# Autodesk Inventor assembly: Drivebox_MIR
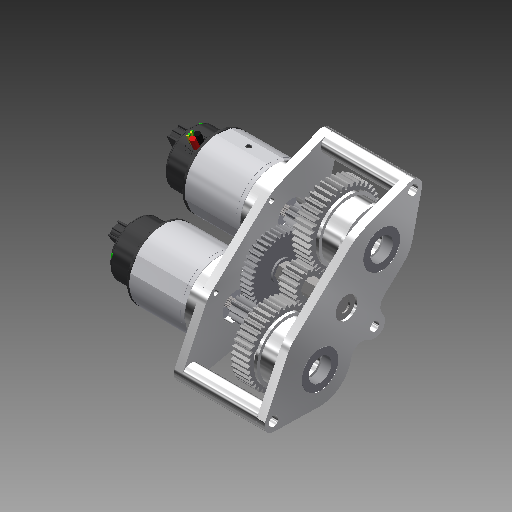
[picture p0: Inventor's stored thumbnail of the model, 512x512]
Saved by Autodesk Inventor 2019.4 (Build 234330000, 330)
## iProperties
Created: 2020-01-05
Part Number: Drivebox_MIR
Document SubType Name: Assembly
Designer: Mark
Mass: 1559.59 g
Surface Area: 2473.44 cm^2
Volume: 631.167 cm^3
Density: 2.47097 g/cm^3
Author: Mark
## Documents named in this file (14)
- C:\Users\admin\Desktop\FRC 2020 Engineering\GitHub\7738-2020\CAD\Gearbox\Drivebox_MIR.iam
- C:\Users\admin\Desktop\FRC 2020 Engineering\GitHub\7738-2020\CAD\Gearbox\Gearbox Plate 1_MIR.ipt
- C:\Users\admin\Desktop\FRC 2020 Engineering\GitHub\7738-2020\CAD\Gearbox\Gearbox Plate 2_MIR.ipt
- C:\Users\admin\Desktop\FRC 2020 Engineering\GitHub\7738-2020\CAD\Gearbox\Shaft Jr_MIR.ipt
- C:\Users\admin\Desktop\FRC 2020 Engineering\GitHub\7738-2020\CAD\Gearbox\F6800_MIR.ipt
- C:\Users\admin\Desktop\FRC 2020 Engineering\GitHub\7738-2020\CAD\Gearbox\Spacer_MIR.ipt
- C:\Users\admin\Desktop\FRC 2020 Engineering\GitHub\7738-2020\CAD\Gearbox\Falcon_500_Powered_by_Talon_FX_217-6515_MIR.ipt
- C:\Users\admin\Desktop\FRC 2020 Engineering\GitHub\7738-2020\CAD\Gearbox\F6804_MIR.ipt
- C:\Users\admin\Desktop\FRC 2020 Engineering\GitHub\7738-2020\CAD\Gearbox\10T_Steel_Spur_Gear_20_DP_12T_Center_Distance_Falcon_Motor_217-6917_MIR.ipt
- C:\Users\admin\Desktop\FRC 2020 Engineering\GitHub\7738-2020\CAD\Gearbox\40t_Aluminum_Spur_Gear_20_DP_1_2_Hex_Bore_217-2708_MIR.ipt
- C:\Users\admin\Desktop\FRC 2020 Engineering\GitHub\7738-2020\CAD\Gearbox\Gearbox\Design Accelerator\Spur Gears1_MIR1.iam
- C:\Users\admin\Desktop\FRC 2020 Engineering\GitHub\7738-2020\CAD\Gearbox\Gearbox\Design Accelerator\Spur Gears2_MIR1.iam
- C:\Users\admin\Desktop\FRC 2020 Engineering\GitHub\7738-2020\CAD\Gearbox\HTD 5M 30 20mm ID Keyed_MIR.ipt
- C:\Users\admin\Desktop\FRC 2020 Engineering\GitHub\7738-2020\CAD\Motor Spacer_MIR.ipt
## Components (21 placed, 13 different names)
1. Gearbox Plate 1_MIR:1 — Flush:3, Mate:4, Mate:3, Mate:45, Mate:47, Mate:46, Mate:14, Mate:13, Mate:18, Mate:17, Mate:16, Mate:15, Mate:25, Mate:26, Mate:43, Mate:54, Mate:56
2. Gearbox Plate 2_MIR:1 — Flush:3, Mate:39, Mate:38, Mate:37, Mate:44, Mate:34, Mate:33, Mate:36, Mate:35, Mate:40, Mate:49, Mate:51
3. Shaft Jr_MIR:1 — Mate:8, Mate:7, Mate:41
4. F6800_MIR:1 — Mate:39, Mate:8, Mate:7, Mate:4, Mate:3, Mate:42
5. F6800_MIR:2 — Mate:41, Mate:38, Mate:37
6. Spacer_MIR:1 — Mate:44, Mate:45
7. Spacer_MIR:2 — Mate:47, Mate:46
8. Spacer_MIR:3 — Mate:14, Mate:13
9. Falcon_500_Powered_by_Talon_FX_217-6515_MIR:1 — Mate:18, Mate:17, Mate:23, Mate:53
10. Falcon_500_Powered_by_Talon_FX_217-6515_MIR:2 — Mate:16, Mate:15, Mate:52, Mate:55
11. F6804_MIR:1 — Mate:34, Mate:33, Mate:31, Mate:50
12. F6804_MIR:2 — Mate:36, Mate:35, Mate:32, Mate:48
13. 10T_Steel_Spur_Gear_20_DP_12T_Center_Distance_Falcon_Motor_217-6917_MIR:1 — Mate:52, Mate:25
14. 10T_Steel_Spur_Gear_20_DP_12T_Center_Distance_Falcon_Motor_217-6917_MIR:2 — Mate:26, Mate:23
15. 40t_Aluminum_Spur_Gear_20_DP_1_2_Hex_Bore_217-2708_MIR:1 — Mate:43, Mate:42, Mate:30
16. Spur Gears1_MIR1:1 [sub-assembly] — Mate:40, Mate:31, Mate:30, Flush:2
17. Spur Gears2_MIR1:1 [sub-assembly] — Flush:2, Mate:32
18. HTD 5M 30 20mm ID Keyed_MIR:1 — Mate:49, Mate:48
19. HTD 5M 30 20mm ID Keyed_MIR:2 — Mate:51, Mate:50
20. Motor Spacer_MIR:1 — Mate:54, Mate:53
21. Motor Spacer_MIR:2 — Mate:56, Mate:55
## Relationships (42: Mate 40, Flush 2)
- Flush:3: Gearbox Plate 1_MIR:1 ↔ Gearbox Plate 2_MIR:1
- Mate:39: Gearbox Plate 2_MIR:1 ↔ F6800_MIR:1
- Mate:8 (0.2 mm): Shaft Jr_MIR:1 ↔ F6800_MIR:1
- Mate:7: Shaft Jr_MIR:1 ↔ F6800_MIR:1
- Mate:4: Gearbox Plate 1_MIR:1 ↔ F6800_MIR:1
- Mate:3: Gearbox Plate 1_MIR:1 ↔ F6800_MIR:1
- Mate:41 (0.2 mm): Shaft Jr_MIR:1 ↔ F6800_MIR:2
- Mate:38: Gearbox Plate 2_MIR:1 ↔ F6800_MIR:2
- Mate:37: Gearbox Plate 2_MIR:1 ↔ F6800_MIR:2
- Mate:44: Gearbox Plate 2_MIR:1 ↔ Spacer_MIR:1
- Mate:45: Gearbox Plate 1_MIR:1 ↔ Spacer_MIR:1
- Mate:47: Gearbox Plate 1_MIR:1 ↔ Spacer_MIR:2
- Mate:46: Gearbox Plate 1_MIR:1 ↔ Spacer_MIR:2
- Mate:14: Gearbox Plate 1_MIR:1 ↔ Spacer_MIR:3
- Mate:13: Gearbox Plate 1_MIR:1 ↔ Spacer_MIR:3
- Mate:18 (7.5 mm): Gearbox Plate 1_MIR:1 ↔ Falcon_500_Powered_by_Talon_FX_217-6515_MIR:1
- Mate:17: Gearbox Plate 1_MIR:1 ↔ Falcon_500_Powered_by_Talon_FX_217-6515_MIR:1
- Mate:16 (7.5 mm): Gearbox Plate 1_MIR:1 ↔ Falcon_500_Powered_by_Talon_FX_217-6515_MIR:2
- Mate:15: Gearbox Plate 1_MIR:1 ↔ Falcon_500_Powered_by_Talon_FX_217-6515_MIR:2
- Mate:34: Gearbox Plate 2_MIR:1 ↔ F6804_MIR:1
- Mate:33: Gearbox Plate 2_MIR:1 ↔ F6804_MIR:1
- Mate:36: Gearbox Plate 2_MIR:1 ↔ F6804_MIR:2
- Mate:35: Gearbox Plate 2_MIR:1 ↔ F6804_MIR:2
- Mate:52: Falcon_500_Powered_by_Talon_FX_217-6515_MIR:2 ↔ 10T_Steel_Spur_Gear_20_DP_12T_Center_Distance_Falcon_Motor_217-6917_MIR:1
- Mate:25 (1 mm): Gearbox Plate 1_MIR:1 ↔ 10T_Steel_Spur_Gear_20_DP_12T_Center_Distance_Falcon_Motor_217-6917_MIR:1
- Mate:26 (1 mm): Gearbox Plate 1_MIR:1 ↔ 10T_Steel_Spur_Gear_20_DP_12T_Center_Distance_Falcon_Motor_217-6917_MIR:2
- Mate:23: Falcon_500_Powered_by_Talon_FX_217-6515_MIR:1 ↔ 10T_Steel_Spur_Gear_20_DP_12T_Center_Distance_Falcon_Motor_217-6917_MIR:2
- Mate:43 (4 mm): Gearbox Plate 1_MIR:1 ↔ 40t_Aluminum_Spur_Gear_20_DP_1_2_Hex_Bore_217-2708_MIR:1
- Mate:42: F6800_MIR:1 ↔ 40t_Aluminum_Spur_Gear_20_DP_1_2_Hex_Bore_217-2708_MIR:1
- Mate:40: Gearbox Plate 2_MIR:1 ↔ Spur Gears1_MIR1:1
- Mate:31: F6804_MIR:1 ↔ Spur Gears1_MIR1:1
- Mate:30 (8 mm): 40t_Aluminum_Spur_Gear_20_DP_1_2_Hex_Bore_217-2708_MIR:1 ↔ Spur Gears1_MIR1:1
- Flush:2: Spur Gears1_MIR1:1 ↔ Spur Gears2_MIR1:1
- Mate:32: F6804_MIR:2 ↔ Spur Gears2_MIR1:1
- Mate:49 (3 mm): Gearbox Plate 2_MIR:1 ↔ HTD 5M 30 20mm ID Keyed_MIR:1
- Mate:48: F6804_MIR:2 ↔ HTD 5M 30 20mm ID Keyed_MIR:1
- Mate:51 (3 mm): Gearbox Plate 2_MIR:1 ↔ HTD 5M 30 20mm ID Keyed_MIR:2
- Mate:50: F6804_MIR:1 ↔ HTD 5M 30 20mm ID Keyed_MIR:2
- Mate:54: Gearbox Plate 1_MIR:1 ↔ Motor Spacer_MIR:1
- Mate:53: Falcon_500_Powered_by_Talon_FX_217-6515_MIR:1 ↔ Motor Spacer_MIR:1
- Mate:56: Gearbox Plate 1_MIR:1 ↔ Motor Spacer_MIR:2
- Mate:55: Falcon_500_Powered_by_Talon_FX_217-6515_MIR:2 ↔ Motor Spacer_MIR:2
